# Autodesk Inventor assembly: smol-gear-stack
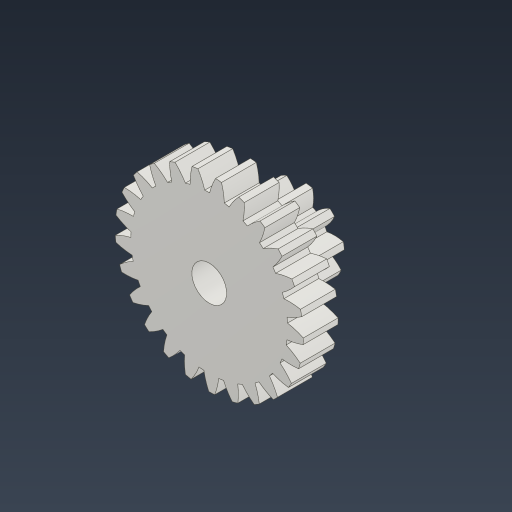
[picture p0: Inventor's stored thumbnail of the model, 512x512]
Saved by Autodesk Inventor 2023 (Build 270158000, 158)
## iProperties
Created: 2025-04-01
Part Number: smol-gear-stack
Document SubType Name: Assembly
Designer: szymo
Author: szymo
## Documents named in this file (3)
- D:\tech\robotyka\robots\evangelion\inventor-project\smol-gear-stack.iam
- D:\tech\robotyka\robots\evangelion\inventor-project\Gears\Design Accelerator\Przekładnia walcowa22.ipt
- D:\tech\robotyka\robots\evangelion\inventor-project\Gears\Design Accelerator\Przekładnia walcowa12.ipt
## Components (2 placed, 2 different names)
1. Przekładnia walcowa1:1 — Mate:1, Mate:2, Mate:3
2. Przekładnia walcowa2:1 — Mate:1, Mate:2, Mate:3
## Relationships (3: Mate 3)
- Mate:1: Przekładnia walcowa1:1 ↔ Przekładnia walcowa2:1
- Mate:2: Przekładnia walcowa1:1 ↔ Przekładnia walcowa2:1
- Mate:3: Przekładnia walcowa1:1 ↔ Przekładnia walcowa2:1
